# Autodesk Inventor assembly: road axle
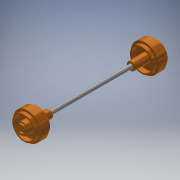
[picture p0: Inventor's stored thumbnail of the model, 180x180]
Saved by Autodesk Inventor 2019.1 (Build 231200000, 200)
## iProperties
Created: 2019-03-15
Part Number: road axle
Document SubType Name: Assembly
Designer: poryz
Author: poryz
## Documents named in this file (4)
- E:\Dropbox\_PRACA\HARDWARE\IE-TRACK-KIT-PWR-1\MECH\wheels\road axle.iam
- E:\Dropbox\_PRACA\HARDWARE\IE-TRACK-KIT-PWR-1\MECH\wheels\3mm shaft.ipt
- E:\Dropbox\_PRACA\HARDWARE\IE-TRACK-KIT-PWR-1\MECH\wheels\hub.ipt
- E:\Dropbox\_PRACA\HARDWARE\IE-TRACK-KIT-PWR-1\MECH\wheels\road wheel.ipt
## Components (5 placed, 3 different names)
1. 3mm shaft:1 — Mate:1, Mate:2, Mate:3, Mate:4, Mate:5, Mate:6
2. hub:1 — Mate:1, Mate:4, Mate:7
3. hub:2 — Mate:2, Mate:3, Mate:8
4. road wheel:1 — Mate:5, Mate:8
5. road wheel:2 — Mate:6, Mate:7
## Relationships (8: Mate 8)
- Mate:1: 3mm shaft:1 ↔ hub:1
- Mate:2: 3mm shaft:1 ↔ hub:2
- Mate:3: 3mm shaft:1 ↔ hub:2
- Mate:4: 3mm shaft:1 ↔ hub:1
- Mate:5: 3mm shaft:1 ↔ road wheel:1
- Mate:6: 3mm shaft:1 ↔ road wheel:2
- Mate:7: hub:1 ↔ road wheel:2
- Mate:8: hub:2 ↔ road wheel:1
